# Autodesk Inventor assembly: STEFAN_2.0
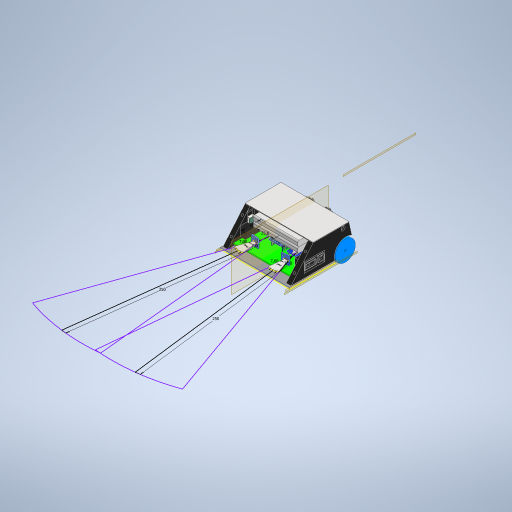
[picture p0: Inventor's stored thumbnail of the model, 512x512]
Saved by Autodesk Inventor 2023 (Build 270158000, 158)
## iProperties
Created: 2023-04-05
Part Number: STEFAN_2.0
Document SubType Name: Assembly
Designer: Kamil
Author: Kamil
## Documents named in this file (19)
- C:\Users\Kamil\Desktop\MojeRoboty\Stefan\mechanics\STEFAN_PRE_2.0 — kopia.iam
- C:\Users\Kamil\Desktop\MojeRoboty\Stefan\mechanics\n20 motor.ipt
- C:\Users\Kamil\Desktop\MojeRoboty\Stefan\mechanics\minisumopodsr.ipt
- C:\Users\Kamil\Desktop\MojeRoboty\Stefan\mechanics\SCIANA_2.0_MIR.ipt
- C:\Users\Kamil\Desktop\MojeRoboty\Stefan\mechanics\PCB.ipt
- C:\Users\Kamil\Desktop\MojeRoboty\Stefan\mechanics\GP2Y0A41SK0F.ipt
- C:\Users\Kamil\Desktop\MojeRoboty\Stefan\mechanics\motor drive module TB6612.ipt
- C:\Users\Kamil\Desktop\MojeRoboty\Stefan\mechanics\ARDUINO_NANO.ipt
- C:\Users\Kamil\Desktop\MojeRoboty\Stefan\mechanics\TOF_VLCOS.ipt
- C:\Users\Kamil\Desktop\MojeRoboty\Stefan\mechanics\GP2Y0A41SK0F_MIR1.ipt
- C:\Users\Kamil\Desktop\MojeRoboty\Stefan\mechanics\servo_stefan.ipt
- C:\Users\Kamil\Desktop\MojeRoboty\Stefan\mechanics\servo_stefan_MIR.ipt
- C:\Users\Kamil\Desktop\MojeRoboty\Stefan\mechanics\bateria szczurza.ipt
- C:\Users\Kamil\Desktop\MojeRoboty\Stefan\mechanics\opona_nowa.ipt
- C:\Users\Kamil\Desktop\MojeRoboty\Stefan\mechanics\mocowanie_serw.ipt
- C:\Users\Kamil\Desktop\MojeRoboty\Stefan\mechanics\PCBE_2_2.ipt
- C:\Users\Kamil\Desktop\MojeRoboty\Stefan\mechanics\pokrywka.ipt
- C:\Users\Kamil\Desktop\MojeRoboty\Stefan\mechanics\uchwyt_nowy.ipt
- C:\Users\Kamil\Desktop\MojeRoboty\Stefan\mechanics\SCIANA_2.0_MIR_MIR.ipt
## Components (22 placed, 18 different names)
1. n20 motor:2 — Równoległe:4, Równoległe:19
2. minisumopodsr:1 — Równoległe:4, Zestawiające:1, Zestawiające:2, Zestawiające:3, Zestawiające:4, Równoległe:7, Zestawiające:25, Równoległe:26, Symetria:2
3. n20 motor:3 — Równoległe:7, Zestawiające:24, Zestawiające:26
4. SCIANA_2.0_MIR:1 — Zestawiające:21, Symetria:2
5. PCB:1 — Zestawiające:14, Zestawiające:16, Zestawiające:17, Równoległe:13, Równoległe:14
6. GP2Y0A41SK0F:1 — Zestawiające:14
7. motor drive module TB6612:1 — Zestawiające:16
8. ARDUINO_NANO:1 — Zestawiające:17
9. TOF_VLCOS:3 — Równoległe:13
10. TOF_VLCOS:4 — Równoległe:14, Zestawiające:21
11. GP2Y0A41SK0F_MIR1:1
12. servo_stefan:1 — Równoległe:16
13. servo_stefan_MIR:1 — Równoległe:16, Równoległe:23
14. bateria szczurza:1 — Zestawiające:23, Równoległe:17, Równoległe:18
15. bateria szczurza:2 — Zestawiające:23, Równoległe:17, Równoległe:18
16. opona_nowa:1 — Równoległe:19
17. opona_nowa:2 — Zestawiające:24
18. mocowanie_serw:1 — Równoległe:23, Równoległe:24
19. PCBE_2_2:1 — Równoległe:24
20. pokrywka:1
21. uchwyt_nowy:1 — Zestawiające:25, Zestawiające:26, Równoległe:26
22. SCIANA_2.0_MIR_MIR:1
## Relationships (25: Mate 12, Flush 11, Symmetry 2)
- Równoległe:4 [Flush]: n20 motor:2 ↔ minisumopodsr:1
- Zestawiające:1 [Mate]: minisumopodsr:1
- Zestawiające:2 [Mate]: minisumopodsr:1
- Zestawiające:3 [Mate]: minisumopodsr:1
- Zestawiające:4 [Mate]: minisumopodsr:1
- Symetria:1 [Symmetry]
- Równoległe:7 [Flush]: minisumopodsr:1 ↔ n20 motor:3
- Zestawiające:14 [Mate]: PCB:1 ↔ GP2Y0A41SK0F:1
- Zestawiające:16 [Mate]: PCB:1 ↔ motor drive module TB6612:1
- Zestawiające:17 [Mate] (8 mm): PCB:1 ↔ ARDUINO_NANO:1
- Równoległe:13 [Flush]: PCB:1 ↔ TOF_VLCOS:3
- Równoległe:14 [Flush]: PCB:1 ↔ TOF_VLCOS:4
- Zestawiające:21 [Mate] (25 mm): SCIANA_2.0_MIR:1 ↔ TOF_VLCOS:4
- Równoległe:16 [Flush]: servo_stefan:1 ↔ servo_stefan_MIR:1
- Zestawiające:23 [Mate]: bateria szczurza:1 ↔ bateria szczurza:2
- Równoległe:17 [Flush]: bateria szczurza:1 ↔ bateria szczurza:2
- Równoległe:18 [Flush]: bateria szczurza:1 ↔ bateria szczurza:2
- Równoległe:19 [Flush]: n20 motor:2 ↔ opona_nowa:1
- Zestawiające:24 [Mate]: n20 motor:3 ↔ opona_nowa:2
- Równoległe:23 [Flush]: servo_stefan_MIR:1 ↔ mocowanie_serw:1
- Równoległe:24 [Flush]: mocowanie_serw:1 ↔ PCBE_2_2:1
- Zestawiające:25 [Mate]: minisumopodsr:1 ↔ uchwyt_nowy:1
- Zestawiające:26 [Mate]: n20 motor:3 ↔ uchwyt_nowy:1
- Równoległe:26 [Flush]: minisumopodsr:1 ↔ uchwyt_nowy:1
- Symetria:2 [Symmetry]: minisumopodsr:1 ↔ SCIANA_2.0_MIR:1
